# Autodesk Inventor assembly: wheel_block
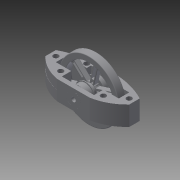
[picture p0: Inventor's stored thumbnail of the model, 180x180]
Saved by Autodesk Inventor 2015 (Build 190159000, 159)
## iProperties
Created: 2015-07-19
Part Number: wheel_block
Document SubType Name: Assembly
Designer: astralien3000
Author: astralien3000
## Documents named in this file (3)
- C:\Users\astralien3000\Desktop\ceres\meca\v2016\wheel_block.iam
- C:\Users\astralien3000\Desktop\ceres\meca\v2016\wheel_base_asm.iam
- C:\Users\astralien3000\Desktop\ceres\meca\v2016\wheel.iam
## Components (2 placed, 2 different names)
1. wheel_base_asm:1 [sub-assembly] — Placage:1, Placage:2, Placage:4, Placage:5, Placage:6
2. wheel:1 [sub-assembly] — Placage:2, Placage:6
## Relationships (5: Mate 5)
- Placage:1 [Mate]: wheel_base_asm:1
- Placage:2 [Mate]: wheel_base_asm:1 ↔ wheel:1
- Placage:4 [Mate]: wheel_base_asm:1
- Placage:5 [Mate]: wheel_base_asm:1
- Placage:6 [Mate] (0.5 mm): wheel_base_asm:1 ↔ wheel:1
